# Autodesk Inventor assembly: montagem cxv2 and painel 1U
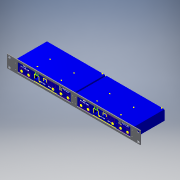
[picture p0: Inventor's stored thumbnail of the model, 180x180]
Saved by Autodesk Inventor 2016 (Build 200138000, 138)
## iProperties
Created: 2015-09-14
Part Number: montagem cxv2 and painel 1U
Document SubType Name: Assembly
Designer: fernando.santanna
Author: fernando.santanna
## Documents named in this file (3)
- D:\bkp\CNPEM\Front-End\Caixa v2\montagem cxv2 and painel 1U.iam
- D:\bkp\CNPEM\Front-End\Caixa v2\1U 19pol 3mm painel.ipt
- D:\bkp\CNPEM\Front-End\Caixa v2\caixa frontend_ serigrafia V2_4.ipt
## Components (3 placed, 2 different names)
1. 1U 19pol 3mm painel:1 — Mate:2, Flush:3, Flush:4
2. caixa frontend_ serigrafia V2_4:1 — Flush:1, Mate:1, Flush:2, Mate:2, Flush:3, Flush:4
3. caixa frontend_ serigrafia V2_4:2 — Flush:1, Mate:1, Flush:2
## Relationships (6: Flush 4, Mate 2)
- Flush:1: caixa frontend_ serigrafia V2_4:1 ↔ caixa frontend_ serigrafia V2_4:2
- Mate:1 (5 mm): caixa frontend_ serigrafia V2_4:1 ↔ caixa frontend_ serigrafia V2_4:2
- Flush:2: caixa frontend_ serigrafia V2_4:1 ↔ caixa frontend_ serigrafia V2_4:2
- Mate:2: 1U 19pol 3mm painel:1 ↔ caixa frontend_ serigrafia V2_4:1
- Flush:3 (4.25 mm): 1U 19pol 3mm painel:1 ↔ caixa frontend_ serigrafia V2_4:1
- Flush:4 (28.8 mm): 1U 19pol 3mm painel:1 ↔ caixa frontend_ serigrafia V2_4:1
